# Autodesk Inventor assembly: POM_T5_00_yooo
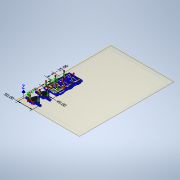
[picture p0: Inventor's stored thumbnail of the model, 180x180]
Saved by Autodesk Inventor 2022 (Build 260153000, 153)
## iProperties
Created: 2022-09-28
Part Number: POM_T5_00_yooo
Document SubType Name: Assembly
Designer: Masato
Author: Masato
## Documents named in this file (5)
- C:\Users\ヨコオリク\Documents\CITBrains\SUSTAINA-OP\Cam\POM_T5\POM_T5_00_yooo.iam
- C:\Users\ヨコオリク\Documents\CITBrains\SUSTAINA-OP\Cam\DisposableBoard.ipt
- C:\Users\ヨコオリク\Documents\CITBrains\SUSTAINA-OP\UpperBody\Head\Camera_side_frame.ipt
- C:\Users\ヨコオリク\Documents\CITBrains\SUSTAINA-OP\UpperBody\Head\Head_horn_frame.ipt
- C:\Users\ヨコオリク\Documents\CITBrains\SUSTAINA-OP\UpperBody\Head\Head_diagonal.ipt
## Components (6 placed, 4 different names)
1. DisposableBoard:1 — フラッシュ:1, フラッシュ:2, フラッシュ:3, フラッシュ:4, メイト:1, メイト:2, メイト:3, メイト:4, メイト:5, メイト:6, メイト:7
2. Head_horn_frame:1 — メイト:4, メイト:5, 正接:1, メイト:8
3. Camera_side_frame:1 — メイト:1, メイト:2, メイト:3
4. Camera_side_frame:2 — 正接:1
5. Head_diagonal:1 — メイト:6, メイト:7, メイト:8
6. Head_diagonal:2
## Component patterns: (2 elements, first: Camera_side_frame:1), (2 elements, first: Head_diagonal:1)
## Relationships (13: Mate 8, Flush 4, Tangent 1)
- フラッシュ:1 [Flush]: DisposableBoard:1
- フラッシュ:2 [Flush]: DisposableBoard:1
- フラッシュ:3 [Flush]: DisposableBoard:1
- フラッシュ:4 [Flush]: DisposableBoard:1
- メイト:1 [Mate]: DisposableBoard:1 ↔ Camera_side_frame:1
- メイト:2 [Mate] (1.5 mm): DisposableBoard:1 ↔ Camera_side_frame:1
- メイト:3 [Mate] (1.5 mm): DisposableBoard:1 ↔ Camera_side_frame:1
- メイト:4 [Mate]: DisposableBoard:1 ↔ Head_horn_frame:1
- メイト:5 [Mate] (1.5 mm): DisposableBoard:1 ↔ Head_horn_frame:1
- 正接:1 [Tangent] (3 mm): Head_horn_frame:1 ↔ Camera_side_frame:2
- メイト:6 [Mate]: DisposableBoard:1 ↔ Head_diagonal:1
- メイト:7 [Mate] (1.5 mm): DisposableBoard:1 ↔ Head_diagonal:1
- メイト:8 [Mate] (3 mm): Head_horn_frame:1 ↔ Head_diagonal:1
